# Autodesk Inventor assembly: Hexagonal Deco Lamp Assembly
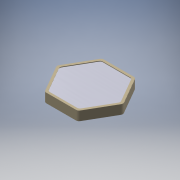
[picture p0: Inventor's stored thumbnail of the model, 180x180]
Saved by Autodesk Inventor 2019 (Build 230136000, 136)
## iProperties
Created: 2021-07-14
Part Number: Hexagonal Deco Lamp Assembly
Document SubType Name: Assembly
Designer: Lix
Author: Lix
## Documents named in this file (4)
- G:\Project\3d-printing\Models\My Own\Hexagonal Deco Lamp\Hexagonal Deco Lamp Assembly.iam
- G:\Project\3d-printing\Models\My Own\Hexagonal Deco Lamp\Frosted Top v1.ipt
- G:\Project\3d-printing\Models\My Own\Hexagonal Deco Lamp\Cover v1.ipt
- G:\Project\3d-printing\Models\My Own\Hexagonal Deco Lamp\Base v2.ipt
## Components (3 placed, 3 different names)
1. Base v2:1 — Flush:2, Flush:3, Mate:5, Flush:4
2. Cover v1:1 — Flush:2, Flush:3, Mate:5, Flush:4, Mate:6, Mate:7, Mate:8
3. Frosted Top v1:1 — Mate:6, Mate:7, Mate:8
## Relationships (7: Mate 4, Flush 3)
- Flush:2: Base v2:1 ↔ Cover v1:1
- Flush:3: Base v2:1 ↔ Cover v1:1
- Mate:5: Base v2:1 ↔ Cover v1:1
- Flush:4: Base v2:1 ↔ Cover v1:1
- Mate:6: Cover v1:1 ↔ Frosted Top v1:1
- Mate:7: Cover v1:1 ↔ Frosted Top v1:1
- Mate:8: Cover v1:1 ↔ Frosted Top v1:1
